# Autodesk Inventor assembly: servo
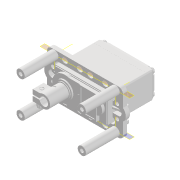
[picture p0: Inventor's stored thumbnail of the model, 180x180]
Saved by Autodesk Inventor 2020 (Build 240168000, 168)
## iProperties
Created: 2019-12-16
Part Number: servo
Document SubType Name: Assembly
Designer: ball
Author: ball
## Documents named in this file (5)
- C:\FTC\FTC8863CAD\2019 Robot\Delivery\extension arm\servo.iam
- C:\FTC\FTC8863CAD\Actobotics\575 parts\575112.ipt
- C:\FTC\FTC8863CAD\Actobotics\633 parts\633130.ipt
- C:\FTC\FTC8863CAD\Actobotics\525 parts\525150 assembly.ipt
- C:\FTC\FTC8863CAD\GoBilda\2000 Parts\2000-0025-0002.ipt
## Components (7 placed, 4 different names)
1. 575112:1 — Mate:1, Mate:2, Flush:1, Mate:5, Mate:6, Mate:7, Mate:8, Mate:9, Mate:10, Mate:11, Mate:12
2. 633130:1 — Mate:7, Mate:8
3. 633130:2 — Mate:11, Mate:12
4. 633130:3 — Mate:5, Mate:6
5. 633130:4 — Mate:9, Mate:10
6. 525150 assembly:1 — Mate:3, Mate:4
7. 2000-0025-0002:1 — Mate:1, Mate:2, Flush:1, Mate:3, Mate:4
## Relationships (13: Mate 12, Flush 1)
- Mate:1: 575112:1 ↔ 2000-0025-0002:1
- Mate:2: 575112:1 ↔ 2000-0025-0002:1
- Flush:1: 575112:1 ↔ 2000-0025-0002:1
- Mate:3: 525150 assembly:1 ↔ 2000-0025-0002:1
- Mate:4: 525150 assembly:1 ↔ 2000-0025-0002:1
- Mate:5: 575112:1 ↔ 633130:3
- Mate:6: 575112:1 ↔ 633130:3
- Mate:7: 575112:1 ↔ 633130:1
- Mate:8: 575112:1 ↔ 633130:1
- Mate:9: 575112:1 ↔ 633130:4
- Mate:10: 575112:1 ↔ 633130:4
- Mate:11: 575112:1 ↔ 633130:2
- Mate:12: 575112:1 ↔ 633130:2
